# Autodesk Inventor assembly: Samolot
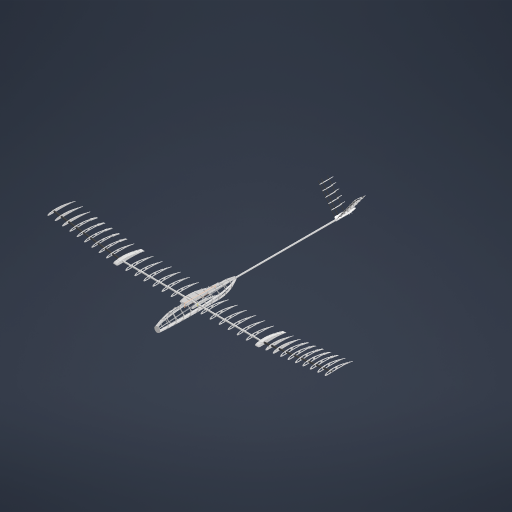
[picture p0: Inventor's stored thumbnail of the model, 512x512]
Saved by Autodesk Inventor 2023 (Build 270158000, 158)
## iProperties
Created: 2023-01-05
Part Number: Samolot
Document SubType Name: Assembly
Designer: szykr
Author: szykr
## Documents named in this file (4)
- D:\Folder Instalacyjny\GitHub Pliki\Solaris\new model\Samolot.iam
- D:\Folder Instalacyjny\GitHub Pliki\Solaris\new model\kadlub_assembly.iam
- D:\Folder Instalacyjny\GitHub Pliki\Solaris\new model\Skrzydło.iam
- D:\Folder Instalacyjny\GitHub Pliki\Solaris\new model\Tail\Tail.iam
## Components (3 placed, 3 different names)
1. kadlub_assembly:1 [sub-assembly] — Flush:1, Mate:1, Mate:2, Insert:1
2. Skrzydło:1 [sub-assembly] — Flush:1, Mate:1, Mate:2
3. Tail:1 [sub-assembly] — Insert:1
## Relationships (4: Mate 2, Flush 1, Insert 1)
- Flush:1: kadlub_assembly:1 ↔ Skrzydło:1
- Mate:1: kadlub_assembly:1 ↔ Skrzydło:1
- Mate:2 (1.227 mm): kadlub_assembly:1 ↔ Skrzydło:1
- Insert:1 (-190 mm): kadlub_assembly:1 ↔ Tail:1
